# Autodesk Inventor assembly: OsnovanieWood
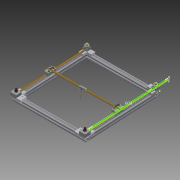
[picture p0: Inventor's stored thumbnail of the model, 180x180]
Saved by Autodesk Inventor 2015 (Build 190159000, 159)
## iProperties
Created: 2016-04-26
Part Number: OsnovanieWood
Document SubType Name: Assembly
Designer: Andreas
Author: Andreas
## Documents named in this file (17)
- C:\Users\Andreas\Documents\GitHub\LaserProject\ласт_ворк_v1.5.3\Sborka.iam
- C:\Users\Andreas\Documents\GitHub\LaserProject\ласт_ворк_v1.5.3\каркас\Balka.ipt
- C:\Users\Andreas\Documents\GitHub\LaserProject\ласт_ворк_v1.5.3\каркас\Ugolok.ipt
- C:\Users\Andreas\Documents\GitHub\LaserProject\ласт_ворк_v1.5.3\каркас\Relsa.ipt
- C:\Users\Andreas\Documents\GitHub\LaserProject\ласт_ворк_v1.5.3\каретка+деталь к ней\Detal+Karetka.iam
- C:\Users\Andreas\Documents\GitHub\LaserProject\ласт_ворк_v1.5.3\мотор\Val.ipt
- C:\Users\Andreas\Documents\GitHub\LaserProject\ласт_ворк_v1.5.3\мотор\Motor.ipt
- C:\Users\Andreas\Documents\GitHub\LaserProject\ласт_ворк_v1.5.3\лазер\Laser.ipt
- C:\Users\Andreas\Documents\GitHub\LaserProject\ласт_ворк_v1.5.3\лазер\ray.ipt
- C:\Users\Andreas\Documents\GitHub\LaserProject\ласт_ворк_v1.5.3\крепление\KreplenieShpon.ipt
- C:\Users\Andreas\Documents\GitHub\LaserProject\ласт_ворк_v1.5.3\новая каретка\NewKaretka.ipt
- C:\Users\Andreas\Documents\GitHub\LaserProject\ласт_ворк_v1.5.3\болты, гайки\bolt3-20.ipt
- C:\Users\Andreas\Documents\GitHub\LaserProject\ласт_ворк_v1.5.3\шпонька\shpon+podship.iam
- C:\Users\Andreas\Documents\GitHub\LaserProject\ласт_ворк_v1.5.3\каркас\UgolokMotor.ipt
- C:\Users\Andreas\Documents\GitHub\LaserProject\ласт_ворк_v1.5.3\каркас\UgolokMotor_MIR.ipt
- C:\Users\Andreas\Documents\GitHub\LaserProject\ласт_ворк_v1.5.3\болты, гайки\gaika3-2.ipt
- C:\Users\Andreas\Documents\GitHub\LaserProject\ласт_ворк_v1.5.3\шпонька\KreplenieBoltam.ipt
## Components (68 placed, 16 different names)
1. Balka:1 — Rigid:1, Rigid:2, Mate:106, Flush:57, Flush:58, Flush:61, Flush:62, Mate:108
2. Balka:2 — Rigid:1, Rigid:3
3. Balka:3 — Rigid:3, Flush:5, Flush:6, Mate:3, Mate:65, Flush:41, Flush:42
4. Balka:4 — Rigid:2
5. Ugolok:3 — Flush:5, Flush:6, Mate:3, Mate:5, Flush:10, Mate:87, Flush:65, Flush:66, Flush:69
6. Ugolok:4 — Mate:65, Flush:41, Flush:42, Mate:86, Flush:67, Flush:68, Mate:110, Flush:70, Flush:71
7. Relsa:1 — Mate:5, Flush:10, Mate:7, Mate:8, Flush:69
8. Relsa:2 — Mate:69, Mate:70, Mate:110, Flush:70, Flush:71
9. Detal+Karetka:1 [sub-assembly] — Mate:7, Mate:8, Flush:22, Flush:23, Mate:22, Flush:24, Mate:98, Tangent:20, Mate:99, Tangent:21, Mate:120, Mate:121
10. Relsa:3 — Flush:23, Mate:22, Flush:24, Mate:96, Mate:97
11. Val:1 — Mate:44, Mate:111
12. Val:2 — Mate:42, Mate:112
13. Motor:1 — Mate:42, Flush:59, Flush:60, Mate:107, Mate:112
14. Motor:2 — Mate:44, Mate:109, Flush:63, Flush:64, Mate:111
15. Laser:1 — Rigid:18, Flush:56, Tangent:19
16. ray:1 — Rigid:18
17. Detal+Karetka:2 [sub-assembly] — Flush:22, Mate:69, Mate:70, Mate:100, Tangent:22, Mate:101, Tangent:23, Mate:115, Mate:117
18. KreplenieShpon:1 — Mate:86, Flush:67, Flush:68, Mate:113, Tangent:28, Mate:118, Mate:152, Mate:153, Mate:154, Mate:155, Tangent:52, Tangent:53, Tangent:54, Tangent:55
19. KreplenieShpon:2 — Mate:87, Flush:65, Flush:66, Mate:114, Tangent:29, Mate:119, Mate:148, Mate:149, Mate:150, Mate:151, Tangent:56, Tangent:57, Tangent:58, Tangent:59
20. NewKaretka:1 — Mate:96, Mate:97, Flush:56, Tangent:19
21. bolt3-20:1 — Mate:98, Tangent:20, Tangent:25, Tangent:33, Tangent:42, Tangent:46, Tangent:48
22. bolt3-20:2 — Mate:99, Tangent:21, Tangent:24, Tangent:32, Tangent:43, Tangent:47, Tangent:49
23. bolt3-20:3 — Mate:100, Tangent:22, Tangent:27, Tangent:30, Tangent:41, Tangent:44, Tangent:51
24. bolt3-20:4 — Mate:113, Tangent:28, Tangent:35, Tangent:36, Tangent:39
25. bolt3-20:7 — Mate:114, Tangent:29, Tangent:34, Tangent:37, Tangent:38
26. bolt3-20:10 — Mate:101, Tangent:23, Tangent:26, Tangent:31, Tangent:40, Tangent:45, Tangent:50
27. shpon+podship:1 [sub-assembly] — Tangent:24, Mate:124, Mate:131
28. shpon+podship:2 [sub-assembly] — Tangent:25, Mate:125, Mate:130
29. shpon+podship:3 [sub-assembly] — Tangent:26, Mate:123, Mate:128
30. shpon+podship:4 [sub-assembly] — Tangent:27, Mate:122, Mate:129
31. UgolokMotor:1 — Mate:106, Flush:57, Flush:58, Flush:59, Flush:60, Mate:107, Mate:140, Mate:141, Mate:142, Mate:143, Tangent:64, Tangent:65, Tangent:66, Tangent:67
32. UgolokMotor_MIR:1 — Flush:61, Flush:62, Mate:108, Mate:109, Flush:63, Flush:64, Mate:144, Mate:145, Mate:146, Mate:147, Tangent:60, Tangent:61, Tangent:62, Tangent:63
33. gaika3-2:1 — Mate:118, Tangent:35, Mate:126
34. gaika3-2:2 — Mate:115, Tangent:30, Mate:122
35. gaika3-2:3 — Mate:117, Tangent:31, Mate:123
36. gaika3-2:4 — Mate:119, Tangent:34, Mate:127
37. gaika3-2:5 — Mate:120, Tangent:32, Mate:124
38. gaika3-2:6 — Mate:121, Tangent:33, Mate:125
39. shpon+podship:5 [sub-assembly] — Mate:126, Tangent:36, Mate:132
40. shpon+podship:6 [sub-assembly] — Tangent:37, Mate:127, Mate:133
41. gaika3-2:7 — Mate:131, Tangent:43
42. gaika3-2:8 — Mate:129, Tangent:41, Mate:134
43. gaika3-2:9 — Mate:130, Tangent:42, Mate:135
44. gaika3-2:10 — Mate:128, Tangent:40
45. gaika3-2:11 — Mate:133, Tangent:38
46. gaika3-2:12 — Mate:132, Tangent:39
47. KreplenieBoltam:1 — Mate:134, Tangent:44, Tangent:45, Mate:136, Mate:137
48. KreplenieBoltam:2 — Mate:135, Tangent:46, Tangent:47, Mate:138, Mate:139
49. gaika3-2:13 — Mate:136, Tangent:51
50. gaika3-2:14 — Mate:137, Tangent:50
51. gaika3-2:15 — Mate:138, Tangent:49
52. gaika3-2:16 — Mate:139, Tangent:48
53. bolt3-20:11 — Mate:148, Tangent:59
54. bolt3-20:12 — Mate:149, Tangent:58
55. bolt3-20:13 — Mate:150, Tangent:56
56. bolt3-20:14 — Mate:151, Tangent:57
57. bolt3-20:15 — Mate:154, Tangent:54
58. bolt3-20:16 — Mate:153, Tangent:52
59. bolt3-20:17 — Mate:152, Tangent:55
60. bolt3-20:18 — Mate:155, Tangent:53
61. bolt3-20:19 — Mate:147, Tangent:62
62. bolt3-20:20 — Mate:146, Tangent:63
63. bolt3-20:21 — Mate:145, Tangent:61
64. bolt3-20:22 — Mate:144, Tangent:60
65. bolt3-20:23 — Mate:143, Tangent:65
66. bolt3-20:24 — Mate:142, Tangent:66
67. bolt3-20:25 — Mate:141, Tangent:67
68. bolt3-20:26 — Mate:140, Tangent:64
## Relationships (144: Mate 67, Tangent 49, Flush 24, WeldJoint 4)
- Rigid:1 [WeldJoint]: Balka:1 ↔ Balka:2
- Rigid:2 [WeldJoint]: Balka:1 ↔ Balka:4
- Rigid:3 [WeldJoint]: Balka:2 ↔ Balka:3
- Flush:5: Balka:3 ↔ Ugolok:3
- Flush:6: Balka:3 ↔ Ugolok:3
- Mate:3: Balka:3 ↔ Ugolok:3
- Mate:5: Ugolok:3 ↔ Relsa:1
- Flush:10 (30 mm): Ugolok:3 ↔ Relsa:1
- Mate:7: Relsa:1 ↔ Detal+Karetka:1
- Mate:8: Relsa:1 ↔ Detal+Karetka:1
- Rigid:18 [WeldJoint]: Laser:1 ↔ ray:1
- Flush:22: Detal+Karetka:1 ↔ Detal+Karetka:2
- Flush:23 (-5 mm): Detal+Karetka:1 ↔ Relsa:3
- Mate:22: Detal+Karetka:1 ↔ Relsa:3
- Flush:24 (25 mm): Detal+Karetka:1 ↔ Relsa:3
- Mate:42: Val:2 ↔ Motor:1
- Mate:44: Val:1 ↔ Motor:2
- Mate:65: Balka:3 ↔ Ugolok:4
- Flush:41: Balka:3 ↔ Ugolok:4
- Flush:42: Balka:3 ↔ Ugolok:4
- Mate:69: Relsa:2 ↔ Detal+Karetka:2
- Mate:70: Relsa:2 ↔ Detal+Karetka:2
- Mate:86: Ugolok:4 ↔ KreplenieShpon:1
- Mate:87: Ugolok:3 ↔ KreplenieShpon:2
- Mate:96: Relsa:3 ↔ NewKaretka:1
- Mate:97: Relsa:3 ↔ NewKaretka:1
- Flush:56: Laser:1 ↔ NewKaretka:1
- Tangent:19: Laser:1 ↔ NewKaretka:1
- Mate:98: Detal+Karetka:1 ↔ bolt3-20:1
- Tangent:20: Detal+Karetka:1 ↔ bolt3-20:1
- Mate:99: Detal+Karetka:1 ↔ bolt3-20:2
- Tangent:21: Detal+Karetka:1 ↔ bolt3-20:2
- Mate:100: Detal+Karetka:2 ↔ bolt3-20:3
- Tangent:22: Detal+Karetka:2 ↔ bolt3-20:3
- Mate:101: Detal+Karetka:2 ↔ bolt3-20:10
- Tangent:23: Detal+Karetka:2 ↔ bolt3-20:10
- Tangent:24: bolt3-20:2 ↔ shpon+podship:1
- Tangent:25: bolt3-20:1 ↔ shpon+podship:2
- Tangent:26: bolt3-20:10 ↔ shpon+podship:3
- Tangent:27: bolt3-20:3 ↔ shpon+podship:4
- Mate:106: Balka:1 ↔ UgolokMotor:1
- Flush:57 (-6 mm): Balka:1 ↔ UgolokMotor:1
- Flush:58: Balka:1 ↔ UgolokMotor:1
- Flush:59: Motor:1 ↔ UgolokMotor:1
- Flush:60: Motor:1 ↔ UgolokMotor:1
- Mate:107: Motor:1 ↔ UgolokMotor:1
- Flush:61 (-16 mm): Balka:1 ↔ UgolokMotor_MIR:1
- Flush:62 (-6 mm): Balka:1 ↔ UgolokMotor_MIR:1
- Mate:108: Balka:1 ↔ UgolokMotor_MIR:1
- Mate:109: Motor:2 ↔ UgolokMotor_MIR:1
- Flush:63: Motor:2 ↔ UgolokMotor_MIR:1
- Flush:64: Motor:2 ↔ UgolokMotor_MIR:1
- Flush:65: Ugolok:3 ↔ KreplenieShpon:2
- Flush:66: Ugolok:3 ↔ KreplenieShpon:2
- Flush:67: Ugolok:4 ↔ KreplenieShpon:1
- Flush:68: Ugolok:4 ↔ KreplenieShpon:1
- Flush:69 (10 mm): Ugolok:3 ↔ Relsa:1
- Mate:110: Ugolok:4 ↔ Relsa:2
- Flush:70 (30 mm): Ugolok:4 ↔ Relsa:2
- Flush:71 (10 mm): Ugolok:4 ↔ Relsa:2
- Mate:111: Val:1 ↔ Motor:2
- Mate:112: Val:2 ↔ Motor:1
- Mate:113: KreplenieShpon:1 ↔ bolt3-20:4
- Tangent:28: KreplenieShpon:1 ↔ bolt3-20:4
- Mate:114: KreplenieShpon:2 ↔ bolt3-20:7
- Tangent:29: KreplenieShpon:2 ↔ bolt3-20:7
- Mate:115: Detal+Karetka:2 ↔ gaika3-2:2
- Tangent:30: bolt3-20:3 ↔ gaika3-2:2
- Mate:117: Detal+Karetka:2 ↔ gaika3-2:3
- Mate:118: KreplenieShpon:1 ↔ gaika3-2:1
- Mate:119: KreplenieShpon:2 ↔ gaika3-2:4
- Mate:120: Detal+Karetka:1 ↔ gaika3-2:5
- Mate:121: Detal+Karetka:1 ↔ gaika3-2:6
- Tangent:31: bolt3-20:10 ↔ gaika3-2:3
- Tangent:32: bolt3-20:2 ↔ gaika3-2:5
- Tangent:33: bolt3-20:1 ↔ gaika3-2:6
- Tangent:34: bolt3-20:7 ↔ gaika3-2:4
- Tangent:35: bolt3-20:4 ↔ gaika3-2:1
- Mate:122: shpon+podship:4 ↔ gaika3-2:2
- Mate:123: shpon+podship:3 ↔ gaika3-2:3
- Mate:124: shpon+podship:1 ↔ gaika3-2:5
- Mate:125: shpon+podship:2 ↔ gaika3-2:6
- Mate:126: gaika3-2:1 ↔ shpon+podship:5
- Tangent:36: bolt3-20:4 ↔ shpon+podship:5
- Tangent:37: bolt3-20:7 ↔ shpon+podship:6
- Mate:127: gaika3-2:4 ↔ shpon+podship:6
- Mate:128: shpon+podship:3 ↔ gaika3-2:10
- Mate:129: shpon+podship:4 ↔ gaika3-2:8
- Mate:130: shpon+podship:2 ↔ gaika3-2:9
- Mate:131: shpon+podship:1 ↔ gaika3-2:7
- Mate:132: shpon+podship:5 ↔ gaika3-2:12
- Mate:133: shpon+podship:6 ↔ gaika3-2:11
- Tangent:38: bolt3-20:7 ↔ gaika3-2:11
- Tangent:39: bolt3-20:4 ↔ gaika3-2:12
- Tangent:40: bolt3-20:10 ↔ gaika3-2:10
- Tangent:41: bolt3-20:3 ↔ gaika3-2:8
- Tangent:42: bolt3-20:1 ↔ gaika3-2:9
- Tangent:43: bolt3-20:2 ↔ gaika3-2:7
- Mate:134: gaika3-2:8 ↔ KreplenieBoltam:1
- Tangent:44: bolt3-20:3 ↔ KreplenieBoltam:1
- Tangent:45: bolt3-20:10 ↔ KreplenieBoltam:1
- Mate:135: gaika3-2:9 ↔ KreplenieBoltam:2
- Tangent:46: bolt3-20:1 ↔ KreplenieBoltam:2
- Tangent:47: bolt3-20:2 ↔ KreplenieBoltam:2
- Mate:136: KreplenieBoltam:1 ↔ gaika3-2:13
- Mate:137: KreplenieBoltam:1 ↔ gaika3-2:14
- Mate:138: KreplenieBoltam:2 ↔ gaika3-2:15
- Mate:139: KreplenieBoltam:2 ↔ gaika3-2:16
- Tangent:48: bolt3-20:1 ↔ gaika3-2:16
- Tangent:49: bolt3-20:2 ↔ gaika3-2:15
- Tangent:50: bolt3-20:10 ↔ gaika3-2:14
- Tangent:51: bolt3-20:3 ↔ gaika3-2:13
- Mate:140: UgolokMotor:1 ↔ bolt3-20:26
- Mate:141: UgolokMotor:1 ↔ bolt3-20:25
- Mate:142: UgolokMotor:1 ↔ bolt3-20:24
- Mate:143: UgolokMotor:1 ↔ bolt3-20:23
- Mate:144: UgolokMotor_MIR:1 ↔ bolt3-20:22
- Mate:145: UgolokMotor_MIR:1 ↔ bolt3-20:21
- Mate:146: UgolokMotor_MIR:1 ↔ bolt3-20:20
- Mate:147: UgolokMotor_MIR:1 ↔ bolt3-20:19
- Mate:148: KreplenieShpon:2 ↔ bolt3-20:11
- Mate:149: KreplenieShpon:2 ↔ bolt3-20:12
- Mate:150: KreplenieShpon:2 ↔ bolt3-20:13
- Mate:151: KreplenieShpon:2 ↔ bolt3-20:14
- Mate:152: KreplenieShpon:1 ↔ bolt3-20:17
- Mate:153: KreplenieShpon:1 ↔ bolt3-20:16
- Mate:154: KreplenieShpon:1 ↔ bolt3-20:15
- Mate:155: KreplenieShpon:1 ↔ bolt3-20:18
- Tangent:52: KreplenieShpon:1 ↔ bolt3-20:16
- Tangent:53: KreplenieShpon:1 ↔ bolt3-20:18
- Tangent:54: KreplenieShpon:1 ↔ bolt3-20:15
- Tangent:55: KreplenieShpon:1 ↔ bolt3-20:17
- Tangent:56: KreplenieShpon:2 ↔ bolt3-20:13
- Tangent:57: KreplenieShpon:2 ↔ bolt3-20:14
- Tangent:58: KreplenieShpon:2 ↔ bolt3-20:12
- Tangent:59: KreplenieShpon:2 ↔ bolt3-20:11
- Tangent:60: UgolokMotor_MIR:1 ↔ bolt3-20:22
- Tangent:61: UgolokMotor_MIR:1 ↔ bolt3-20:21
- Tangent:62: UgolokMotor_MIR:1 ↔ bolt3-20:19
- Tangent:63: UgolokMotor_MIR:1 ↔ bolt3-20:20
- Tangent:64: UgolokMotor:1 ↔ bolt3-20:26
- Tangent:65: UgolokMotor:1 ↔ bolt3-20:23
- Tangent:66: UgolokMotor:1 ↔ bolt3-20:24
- Tangent:67: UgolokMotor:1 ↔ bolt3-20:25
